# Autodesk Inventor assembly: Camera Assembly
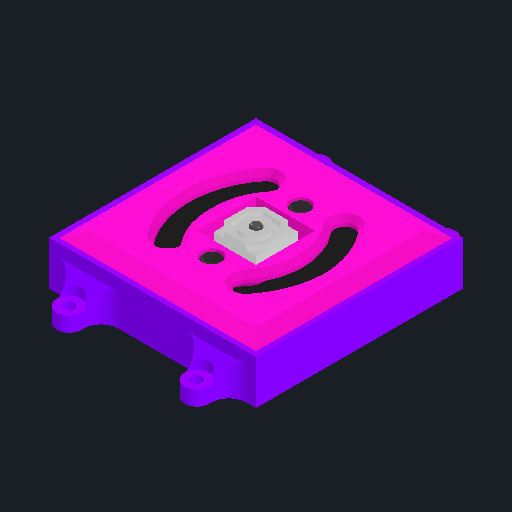
[picture p0: Inventor's stored thumbnail of the model, 512x512]
Saved by Autodesk Inventor 2026 (Build 300175000, 175)
## iProperties
Created: 2024-11-09
Part Number: Camera Assembly
Document SubType Name: Assembly
Designer: jerem
Author: jerem
## Documents named in this file (6)
- C:\Users\jerem\Documents\GitHub\Perovskite-Automated-Synthesis-System\CAD\Camera\Camera Assembly.iam
- C:\Users\jerem\Documents\GitHub\Perovskite-Automated-Synthesis-System\CAD\Camera\CameraMount.ipt
- C:\Users\jerem\Documents\GitHub\Perovskite-Automated-Synthesis-System\CAD\Non 3D Printed Parts\Camera.ipt
- C:\Users\jerem\Documents\GitHub\Perovskite-Automated-Synthesis-System\CAD\Camera\Camera Cover.ipt
- C:\Users\jerem\Documents\GitHub\Perovskite-Automated-Synthesis-System\CAD\Non 3D Printed Parts\Nuts\M2 Nut.ipt
- C:\Users\jerem\Documents\GitHub\Perovskite-Automated-Synthesis-System\CAD\Non 3D Printed Parts\Screws\M2x8.ipt
## Components (7 placed, 5 different names)
1. CameraMount:1 — Mate:1, Mate:2, Mate:3, Mate:9, Mate:10, Angle:1, Angle:2, Flush:1, Flush:2
2. Camera:1 — Mate:1, Mate:2, Mate:3, Mate:6, Mate:7, Mate:8
3. Camera Cover:1 — Mate:6, Mate:7, Mate:8, Mate:11, Mate:12, Mate:13, Mate:14
4. M2 Nut:1 — Mate:10, Angle:1, Flush:1
5. M2 Nut:2 — Mate:9, Angle:2, Flush:2
6. M2x8:1 — Mate:11, Mate:13
7. M2x8:2 — Mate:12, Mate:14
## Relationships (16: Mate 12, Angle 2, Flush 2)
- Mate:1: CameraMount:1 ↔ Camera:1
- Mate:2: CameraMount:1 ↔ Camera:1
- Mate:3: CameraMount:1 ↔ Camera:1
- Mate:6: Camera:1 ↔ Camera Cover:1
- Mate:7: Camera:1 ↔ Camera Cover:1
- Mate:8: Camera:1 ↔ Camera Cover:1
- Mate:9: CameraMount:1 ↔ M2 Nut:2
- Mate:10: CameraMount:1 ↔ M2 Nut:1
- Angle:1 (0 deg): CameraMount:1 ↔ M2 Nut:1
- Angle:2 (0 deg): CameraMount:1 ↔ M2 Nut:2
- Flush:1: CameraMount:1 ↔ M2 Nut:1
- Flush:2: CameraMount:1 ↔ M2 Nut:2
- Mate:11: Camera Cover:1 ↔ M2x8:1
- Mate:12: Camera Cover:1 ↔ M2x8:2
- Mate:13: Camera Cover:1 ↔ M2x8:1
- Mate:14: Camera Cover:1 ↔ M2x8:2
